# Autodesk Inventor assembly: Kettenantrieb
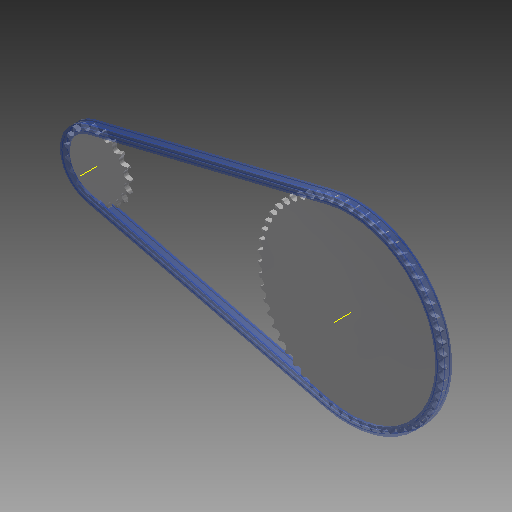
[picture p0: Inventor's stored thumbnail of the model, 512x512]
Saved by Autodesk Inventor 2018 (Build 220112000, 112)
## iProperties
ClientObjectVersion: 1
Created: 2018-01-11
Part Number: Kettenantrieb
Document SubType Name: Assembly
Designer: Dominik
Author: Dominik
## Documents named in this file (4)
- C:\Users\Dominik\Desktop\Diplomarbeit\fuettr_prototype\Mechanical\Inventorskizzen\Kettezusammensetzen\Konstruktions-Assistent\Kettenantrieb1.iam
- C:\Users\Dominik\Desktop\Diplomarbeit\fuettr_prototype\Mechanical\Inventorskizzen\Kettezusammensetzen\Konstruktions-Assistent\Rollenkette1.ipt
- C:\Users\Dominik\Desktop\Diplomarbeit\fuettr_prototype\Mechanical\Inventorskizzen\Kettezusammensetzen\Konstruktions-Assistent\Kettenrad der Rollenkette11.ipt
- C:\Users\Dominik\Desktop\Diplomarbeit\fuettr_prototype\Mechanical\Inventorskizzen\Kettezusammensetzen\Konstruktions-Assistent\Kettenrad der Rollenkette21.ipt
## Components (3 placed, 3 different names)
1. Rollenkette:1 — Fluchtend:1, Passend:1, Passend:2, Fluchtend:2, Passend:3, Passend:4
2. Kettenrad der Rollenkette1:1 — Fluchtend:1, Passend:1, Passend:2, Drehung:1
3. Kettenrad der Rollenkette2:1 — Fluchtend:2, Passend:3, Drehung:1, Passend:4
## Relationships (7: Mate 4, Flush 2, RelateRotation 1)
- Fluchtend:1 [Flush]: Rollenkette:1 ↔ Kettenrad der Rollenkette1:1
- Passend:1 [Mate]: Rollenkette:1 ↔ Kettenrad der Rollenkette1:1
- Passend:2 [Mate]: Rollenkette:1 ↔ Kettenrad der Rollenkette1:1
- Fluchtend:2 [Flush]: Rollenkette:1 ↔ Kettenrad der Rollenkette2:1
- Passend:3 [Mate]: Rollenkette:1 ↔ Kettenrad der Rollenkette2:1
- Drehung:1 [RelateRotation] (3 ul): Kettenrad der Rollenkette1:1 ↔ Kettenrad der Rollenkette2:1
- Passend:4 [Mate]: Rollenkette:1 ↔ Kettenrad der Rollenkette2:1
